# Autodesk Inventor assembly: Сборка3
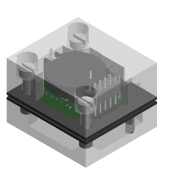
[picture p0: Inventor's stored thumbnail of the model, 180x180]
Saved by Autodesk Inventor 2015 SP1 (Build 190203100, 203)
## iProperties
Created: 2015-12-01
Part Number: Сборка3
Document SubType Name: Assembly
Designer: User
Mass: 31.8846 g
Surface Area: 212.087 cm^2
Volume: 23.0052 cm^3
Density: 1.38597 g/cm^3
Author: User
Title: external
## Documents named in this file (14)
- G:\Mihail\Documents\kurs_mark\DipTrace\Imported Components\fuel_level_1h\Сборка3.iam
- G:\Mihail\Documents\kurs_mark\DipTrace\Imported Components\fuel_level_1h\conn_sensor.ipt
- G:\Mihail\Documents\kurs_mark\DipTrace\Imported Components\fuel_level_1h\button.ipt
- G:\Mihail\Documents\kurs_mark\DipTrace\Imported Components\fuel_level_1h\Imported Components\fuel_level_1h2\fuel_level_1h2.iam
- G:\Mihail\Documents\kurs_mark\DipTrace\Imported Components\fuel_level_1h\case_top.ipt
- G:\Mihail\Documents\kurs_mark\DipTrace\Imported Components\fuel_level_1h\bs-7.ipt
- G:\Mihail\Documents\kurs_mark\DipTrace\Imported Components\fuel_level_1h\hdr-2x5t_2.54x2.54_13x5.ipt
- G:\Mihail\Documents\kurs_mark\DipTrace\Imported Components\fuel_level_1h\MOLEX.ipt
- G:\Mihail\Documents\kurs_mark\DipTrace\Imported Components\fuel_level_1h\jumper.ipt
- G:\Mihail\Documents\kurs_mark\DipTrace\Imported Components\fuel_level_1h\case_bottom.ipt
- G:\Mihail\Documents\kurs_mark\DipTrace\Imported Components\fuel_level_1h\resin_bottom.ipt
- G:\Mihail\Documents\kurs_mark\DipTrace\Imported Components\fuel_level_1h\resin_top.ipt
- G:\Mihail\Documents\kurs_mark\DipTrace\Imported Components\fuel_level_1h\bonka.ipt
- G:\Mihail\Documents\kurs_mark\DipTrace\Imported Components\fuel_level_1h\screw_M3-16.ipt
## Components (17 placed, 13 different names)
1. conn_sensor:1 — Жесткий:2
2. button:1 — Жесткий:3
3. fuel_level_1h2:1 [sub-assembly] — Жесткий:2, Жесткий:3, Заподлицо:3, Заподлицо:4
4. case_top:1 — Цилиндрический:1, Жесткий:6, Rigid:7, Rigid:8, Rigid:9
5. bs-7:1 — Совмещение:1
6. hdr-2x5t_2.54x2.54_13x5:1
7. MOLEX:1 — Совмещение:1, Заподлицо:4, Заподлицо:5, Совмещение:2
8. jumper:1 — Заподлицо:5
9. case_bottom:1 — Совмещение:2, Цилиндрический:1, Rigid:10, Rigid:11, Rigid:12
10. resin_bottom:1
11. resin_top:1 — Жесткий:6
12. bonka:1 — Rigid:7
13. bonka:2 — Rigid:8
14. bonka:3 — Rigid:9
15. screw_M3-16:1 — Rigid:12
16. screw_M3-16:2 — Rigid:11
17. screw_M3-16:3 — Rigid:10
## Relationships (15: WeldJoint 9, Flush 3, Mate 2, CylindricalJoint 1)
- Жесткий:2 [WeldJoint] (0.3 mm): conn_sensor:1 ↔ fuel_level_1h2:1
- Жесткий:3 [WeldJoint]: button:1 ↔ fuel_level_1h2:1
- Совмещение:1 [Mate]: bs-7:1 ↔ MOLEX:1
- Заподлицо:3 [Flush]: fuel_level_1h2:1
- Заподлицо:4 [Flush] (-11 mm): fuel_level_1h2:1 ↔ MOLEX:1
- Заподлицо:5 [Flush]: MOLEX:1 ↔ jumper:1
- Совмещение:2 [Mate]: MOLEX:1 ↔ case_bottom:1
- Цилиндрический:1 [CylindricalJoint]: case_top:1 ↔ case_bottom:1
- Жесткий:6 [WeldJoint]: case_top:1 ↔ resin_top:1
- Rigid:7 [WeldJoint]: case_top:1 ↔ bonka:1
- Rigid:8 [WeldJoint]: case_top:1 ↔ bonka:2
- Rigid:9 [WeldJoint]: case_top:1 ↔ bonka:3
- Rigid:10 [WeldJoint]: case_bottom:1 ↔ screw_M3-16:3
- Rigid:11 [WeldJoint]: case_bottom:1 ↔ screw_M3-16:2
- Rigid:12 [WeldJoint]: case_bottom:1 ↔ screw_M3-16:1
